# Autodesk Inventor assembly: lever_group
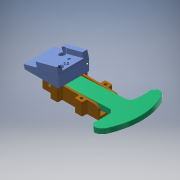
[picture p0: Inventor's stored thumbnail of the model, 180x180]
Saved by Autodesk Inventor 2019 (Build 230136000, 136)
## iProperties
Created: 2021-01-29
Part Number: lever_group
Material: Genérico
Document SubType Name: Assembly
Designer: Juan M. Casillas
Author: Juan M. Casillas
## Documents named in this file (5)
- K:\3DPrinting\3DModels\shifter\lever_group.iam
- K:\3DPrinting\3DModels\shifter\base_plate.ipt
- K:\3DPrinting\3DModels\shifter\lever.ipt
- K:\3DPrinting\3DModels\shifter\cap.ipt
- K:\3DPrinting\3DModels\shifter\microswitch.ipt
## Components (4 placed, 4 different names)
1. base_plate:1 — Rotational:1, Rigid:1, Rigid:2
2. lever:1 — Rotational:1
3. cap:1 — Rigid:1
4. microswitch:1 — Rigid:2
## Relationships (3: WeldJoint 2, RevoluteJoint 1)
- Rotational:1 [RevoluteJoint] (0.5 mm): base_plate:1 ↔ lever:1
- Rigid:1 [WeldJoint]: base_plate:1 ↔ cap:1
- Rigid:2 [WeldJoint] (0.5 mm): base_plate:1 ↔ microswitch:1
